# Autodesk Inventor assembly: AssemblyRespiratoriam
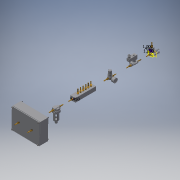
[picture p0: Inventor's stored thumbnail of the model, 180x180]
Saved by Autodesk Inventor 2018 (Build 220112000, 112)
## iProperties
Created: 2020-03-29
Part Number: AssemblyRespiratoriam
Document SubType Name: Assembly
Designer: emile
Author: emile
## Documents named in this file (7)
- C:\Users\emile\OneDrive\Documents\GitHub\VentilatorCovid19\Respirator\MultiLine\AssemblyRespiratoriam.iam
- C:\Users\emile\OneDrive\Documents\GitHub\VentilatorCovid19\Respirator\MultiLine\SolenoidValve.iam
- C:\Users\emile\OneDrive\Documents\GitHub\VentilatorCovid19\Respirator\MultiLine\Air filter.iam
- C:\Users\emile\OneDrive\Documents\GitHub\VentilatorCovid19\Respirator\MultiLine\Pressure regulator.iam
- C:\Users\emile\OneDrive\Documents\GitHub\VentilatorCovid19\Respirator\MultiLine\WaterOilSeparator.iam
- C:\Users\emile\OneDrive\Documents\GitHub\VentilatorCovid19\Respirator\MultiLine\SplitterBlock.iam
- C:\Users\emile\OneDrive\Documents\GitHub\VentilatorCovid19\Respirator\Peep\AirPressure\PeepVavle.iam
## Components (6 placed, 6 different names)
1. SolenoidValve:1 [sub-assembly] — Mate:3, Angle:3, Mate:8, Mate:9, Mate:10
2. Air filter:1 [sub-assembly] — Mate:4, Mate:6
3. Pressure regulator:1 [sub-assembly] — Mate:2, Mate:3, Flush:1, Flush:2, Mate:7, Mate:8
4. WaterOilSeparator:1 [sub-assembly] — Mate:1, Mate:4, Angle:2, Mate:5, Mate:6
5. SplitterBlock:1 [sub-assembly] — Mate:1, Mate:2, Angle:1, Mate:5, Mate:7
6. PeepVavle:1 [sub-assembly] — Mate:9, Mate:10, Angle:4
## Relationships (16: Mate 10, Angle 4, Flush 2)
- Mate:1: WaterOilSeparator:1 ↔ SplitterBlock:1
- Mate:2: Pressure regulator:1 ↔ SplitterBlock:1
- Mate:3: SolenoidValve:1 ↔ Pressure regulator:1
- Mate:4: Air filter:1 ↔ WaterOilSeparator:1
- Flush:1: Pressure regulator:1
- Flush:2: Pressure regulator:1
- Angle:1 (0 deg): SplitterBlock:1
- Angle:2 (0 deg): WaterOilSeparator:1
- Angle:3 (0 deg): SolenoidValve:1
- Mate:5 (50.8 mm): WaterOilSeparator:1 ↔ SplitterBlock:1
- Mate:6 (101.6 mm): Air filter:1 ↔ WaterOilSeparator:1
- Mate:7 (101.6 mm): Pressure regulator:1 ↔ SplitterBlock:1
- Mate:8 (101.6 mm): SolenoidValve:1 ↔ Pressure regulator:1
- Mate:9: SolenoidValve:1 ↔ PeepVavle:1
- Mate:10 (50.8 mm): SolenoidValve:1 ↔ PeepVavle:1
- Angle:4 (180 deg): PeepVavle:1
